# Autodesk Inventor assembly: ImpellerAssembly
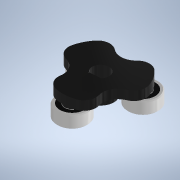
[picture p0: Inventor's stored thumbnail of the model, 180x180]
Saved by Autodesk Inventor 2020.2 (Build 242310000, 310)
## iProperties
Created: 2020-09-03
Part Number: ImpellerAssembly
Document SubType Name: Assembly
Designer: JK
Author: JK
## Documents named in this file (3)
- C:\Users\JK\Documents\Inventor\PeristalticPump\ImpellerAssembly.iam
- C:\Users\JK\Documents\Inventor\PeristalticPump\Impeller.ipt
- C:\Users\JK\Documents\Inventor\PeristalticPump\623zz.iam
## Components (4 placed, 2 different names)
1. Impeller:1 — Mate:1, Mate:2, Mate:3, Mate:4
2. 623zz:1 [sub-assembly] — Flush:1, Flush:2, Mate:1
3. 623zz:2 [sub-assembly] — Flush:1, Mate:2
4. 623zz:3 [sub-assembly] — Flush:2, Mate:3, Mate:4
## Relationships (6: Mate 4, Flush 2)
- Flush:1: 623zz:1 ↔ 623zz:2
- Flush:2: 623zz:1 ↔ 623zz:3
- Mate:1: Impeller:1 ↔ 623zz:1
- Mate:2: Impeller:1 ↔ 623zz:2
- Mate:3: Impeller:1 ↔ 623zz:3
- Mate:4: Impeller:1 ↔ 623zz:3
